# Autodesk Inventor assembly: Assembly_Opentrons_Autofocus_v0
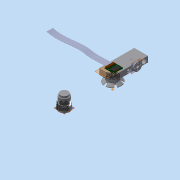
[picture p0: Inventor's stored thumbnail of the model, 180x180]
Saved by Autodesk Inventor 2019.4 (Build 234330000, 330)
## iProperties
Created: 2020-10-23
Part Number: Assembly_Opentrons_Autofocus_v0
Document SubType Name: Assembly
Designer: diederichbenedict
Author: diederichbenedict
## Documents named in this file (10)
- C:\Users\diederichbenedict\Dropbox\Dokumente\Promotion\PROJECTS\OPENTRONS\INVENTOR\Assembly_Opentrons_Autofocus_10x_v0.iam
- C:\Users\diederichbenedict\Dropbox\Dokumente\Promotion\PROJECTS\OPENTRONS\INVENTOR\00_Ringmagnet_25mm.ipt
- C:\Users\diederichbenedict\Dropbox\Dokumente\Promotion\PROJECTS\OPENTRONS\INVENTOR\00_RasPi_Camera.ipt
- C:\Users\diederichbenedict\Dropbox\Dokumente\Promotion\PROJECTS\OPENTRONS\INVENTOR\01_Slide_camera_x_v0.ipt
- C:\Users\diederichbenedict\Dropbox\Dokumente\Promotion\PROJECTS\OPENTRONS\INVENTOR\00_IGUS_Drylin_RJ4JP-01-06.ipt
- C:\Users\diederichbenedict\Dropbox\Dokumente\Promotion\PROJECTS\OPENTRONS\INVENTOR\00_spindel_slide.ipt
- C:\Users\diederichbenedict\Dropbox\Dokumente\Promotion\PROJECTS\OPENTRONS\INVENTOR\00_objectivelens_10x _withoutcap.ipt
- C:\Users\diederichbenedict\Dropbox\Dokumente\Promotion\PROJECTS\OPENTRONS\INVENTOR\01_Autofocus_objecitvelens_10x_spring_1.ipt
- C:\Users\diederichbenedict\Dropbox\Dokumente\Promotion\PROJECTS\OPENTRONS\INVENTOR\01_Autofocus_Magnet_holder_10xobjective_v0.ipt
- C:\Users\diederichbenedict\Dropbox\Dokumente\Promotion\PROJECTS\OPENTRONS\INVENTOR\01_Autofocus_10x_objective_copper_coil.ipt
## Components (14 placed, 9 different names)
1. 00_RasPi_Camera:1 — Angle:2
2. 01_Autofocus_Magnet_holder_10xobjective_v0:1 — Insert:6
3. 00_IGUS_Drylin_RJ4JP-01-06:1
4. 00_spindel_slide:1 — Insert:5
5. 01_Slide_camera_x_v0:1 — Insert:5
6. 01_Autofocus_objecitvelens_10x_spring_1:1 — Mate:1, Flush:5, Flush:6
7. 00_Ringmagnet_25mm:5 — Insert:7
8. 00_Ringmagnet_25mm:6 — Insert:6, Insert:7
9. 00_objectivelens_10x _withoutcap:1 — Insert:8, Mate:1
10. 00_Ringmagnet_25mm:7 — Insert:8, Insert:9
11. 00_Ringmagnet_25mm:9 — Insert:11
12. 00_Ringmagnet_25mm:10 — Insert:10, Insert:11
13. 00_Ringmagnet_25mm:11 — Insert:9, Insert:10
14. 01_Autofocus_10x_objective_copper_coil:1 — Flush:5, Flush:6
## Relationships (12: Insert 7, Flush 3, Angle 1, Mate 1)
- Angle:2 (0 deg): 00_RasPi_Camera:1
- [Flush]: 01_Autofocus_Magnet_holder_10xobjective_v0:1 ↔ 01_Slide_camera_x_v0:1
- Insert:5: 00_spindel_slide:1 ↔ 01_Slide_camera_x_v0:1
- Insert:6: 01_Autofocus_Magnet_holder_10xobjective_v0:1 ↔ 00_Ringmagnet_25mm:6
- Insert:7: 00_Ringmagnet_25mm:5 ↔ 00_Ringmagnet_25mm:6
- Insert:8 (5 mm): 00_objectivelens_10x _withoutcap:1 ↔ 00_Ringmagnet_25mm:7
- Insert:9: 00_Ringmagnet_25mm:7 ↔ 00_Ringmagnet_25mm:11
- Insert:10: 00_Ringmagnet_25mm:10 ↔ 00_Ringmagnet_25mm:11
- Insert:11: 00_Ringmagnet_25mm:9 ↔ 00_Ringmagnet_25mm:10
- Mate:1: 01_Autofocus_objecitvelens_10x_spring_1:1 ↔ 00_objectivelens_10x _withoutcap:1
- Flush:5: 01_Autofocus_objecitvelens_10x_spring_1:1 ↔ 01_Autofocus_10x_objective_copper_coil:1
- Flush:6: 01_Autofocus_objecitvelens_10x_spring_1:1 ↔ 01_Autofocus_10x_objective_copper_coil:1
## Named parameters: d13_d8 = 0 mm
